# Autodesk Inventor assembly: mot_27_ass_MIR
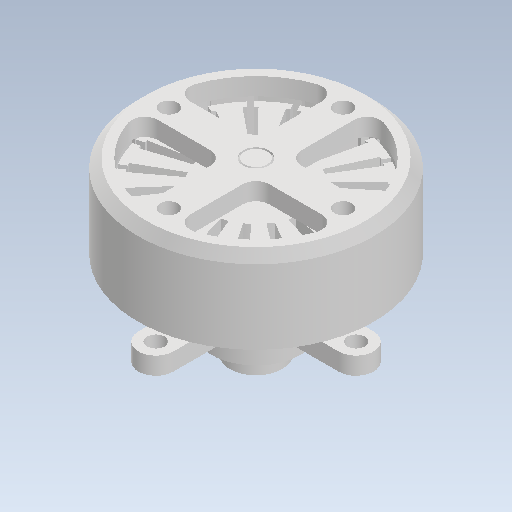
[picture p0: Inventor's stored thumbnail of the model, 512x512]
Saved by Autodesk Inventor 2020 (Build 240168000, 168)
## iProperties
Created: 2020-12-02
Part Number: mot_27_ass_MIR
Document SubType Name: Assembly
Designer: Shuang Peng
Author: Shuang Peng
## Documents named in this file (3)
- D:\projects-3\biped_tiny\hardware\mot_27_ass_MIR.iam
- D:\projects-3\biped_tiny\hardware\mot_27_2_MIR.ipt
- D:\projects-3\biped_tiny\hardware\mot_27_1_MIR.ipt
## Components (2 placed, 2 different names)
1. mot_27_2_MIR:1 — Angle:1, Insert:1
2. mot_27_1_MIR:1 — Angle:1, Insert:1
## Relationships (2: Angle 1, Insert 1)
- Angle:1 (0 deg): mot_27_2_MIR:1 ↔ mot_27_1_MIR:1
- Insert:1: mot_27_2_MIR:1 ↔ mot_27_1_MIR:1
